# Autodesk Inventor assembly: Assembly - Main
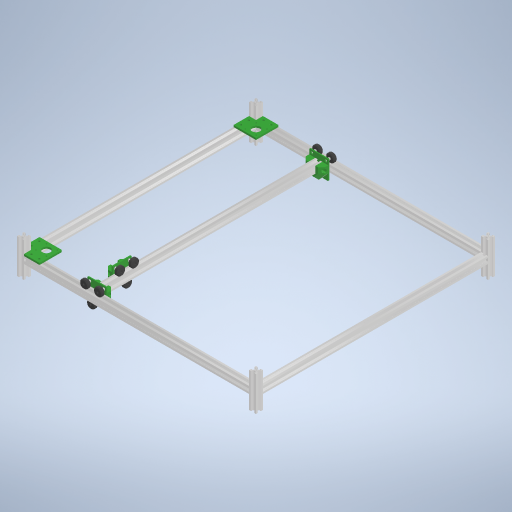
[picture p0: Inventor's stored thumbnail of the model, 512x512]
Saved by Autodesk Inventor 2023 (Build 270158000, 158)
## iProperties
Created: 2023-04-10
Part Number: Assembly - Main
Document SubType Name: Assembly
Designer: ethan
Author: ethan
## Documents named in this file (6)
- C:\Users\ethan\Documents\GitHub\WU-AutomaticChessboard\CAD\Assembly - Main.iam
- C:\Users\ethan\Documents\GitHub\WU-AutomaticChessboard\CAD\VSlot Extrusion 20x20x650mm.ipt
- C:\Users\ethan\Documents\GitHub\WU-AutomaticChessboard\CAD\VSlot Extrusion 20x20x100mm.ipt
- C:\Users\ethan\Documents\GitHub\WU-AutomaticChessboard\CAD\Assembly - GantryPlate.iam
- C:\Users\ethan\Documents\GitHub\WU-AutomaticChessboard\CAD\VSlot Extrusion 20x20x637,50mm.ipt
- C:\Users\ethan\Documents\GitHub\WU-AutomaticChessboard\CAD\NEMA17 Stepper CornerMount.ipt
## Components (14 placed, 5 different names)
1. VSlot Extrusion 20x20x650mm:1 — Flush:1, Mate:1, Flush:2, Flush:5, Mate:3, Flush:6, Flush:15, Tangent:3, Tangent:4, Tangent:6, Flush:22
2. VSlot Extrusion 20x20x650mm:2 — Mate:2, Flush:3, Flush:4, Mate:4, Flush:7, Flush:14
3. VSlot Extrusion 20x20x650mm:3 — Mate:8, Flush:12, Flush:13, Flush:20, Mate:13, Flush:21, Mate:14
4. VSlot Extrusion 20x20x650mm:4 — Mate:6, Flush:8, Flush:9, Mate:7, Flush:10, Flush:11, Mate:9, Tangent:1, Tangent:2, Tangent:5, Flush:19
5. VSlot Extrusion 20x20x100mm:1 — Mate:7, Flush:10, Flush:11, Mate:8, Flush:12, Flush:13
6. VSlot Extrusion 20x20x100mm:2 — Mate:4, Flush:7, Mate:6, Flush:8, Flush:9, Flush:14
7. VSlot Extrusion 20x20x100mm:3 — Flush:5, Mate:3, Flush:6
8. VSlot Extrusion 20x20x100mm:4 — Flush:1, Mate:1, Flush:2, Mate:2, Flush:3, Flush:4
9. Assembly - GantryPlate:1 [sub-assembly] — Mate:9, Tangent:1, Tangent:2, Tangent:5, Mate:12, Flush:17
10. Assembly - GantryPlate:2 [sub-assembly] — Flush:15, Tangent:3, Tangent:4, Tangent:6, Mate:10, Mate:11, Flush:16
11. VSlot Extrusion 20x20x637,50mm:1 — Mate:10, Mate:11, Flush:16, Mate:12, Flush:17, Flush:18, Tangent:7, Tangent:8, Tangent:9
12. Assembly - GantryPlate:3 [sub-assembly] — Flush:18, Tangent:7, Tangent:8, Tangent:9
13. NEMA17 Stepper CornerMount:1 — Flush:19, Flush:20, Mate:13
14. NEMA17 Stepper CornerMount:2 — Flush:21, Flush:22, Mate:14
## Relationships (44: Flush 22, Mate 13, Tangent 9)
- Flush:1: VSlot Extrusion 20x20x650mm:1 ↔ VSlot Extrusion 20x20x100mm:4
- Mate:1: VSlot Extrusion 20x20x650mm:1 ↔ VSlot Extrusion 20x20x100mm:4
- Flush:2 (-40 mm): VSlot Extrusion 20x20x650mm:1 ↔ VSlot Extrusion 20x20x100mm:4
- Mate:2: VSlot Extrusion 20x20x650mm:2 ↔ VSlot Extrusion 20x20x100mm:4
- Flush:3: VSlot Extrusion 20x20x650mm:2 ↔ VSlot Extrusion 20x20x100mm:4
- Flush:4 (-40 mm): VSlot Extrusion 20x20x650mm:2 ↔ VSlot Extrusion 20x20x100mm:4
- Flush:5: VSlot Extrusion 20x20x650mm:1 ↔ VSlot Extrusion 20x20x100mm:3
- Mate:3: VSlot Extrusion 20x20x650mm:1 ↔ VSlot Extrusion 20x20x100mm:3
- Flush:6 (-40 mm): VSlot Extrusion 20x20x650mm:1 ↔ VSlot Extrusion 20x20x100mm:3
- Mate:4: VSlot Extrusion 20x20x650mm:2 ↔ VSlot Extrusion 20x20x100mm:2
- Flush:7: VSlot Extrusion 20x20x650mm:2 ↔ VSlot Extrusion 20x20x100mm:2
- Mate:6: VSlot Extrusion 20x20x650mm:4 ↔ VSlot Extrusion 20x20x100mm:2
- Flush:8: VSlot Extrusion 20x20x650mm:4 ↔ VSlot Extrusion 20x20x100mm:2
- Flush:9 (-40 mm): VSlot Extrusion 20x20x650mm:4 ↔ VSlot Extrusion 20x20x100mm:2
- Mate:7: VSlot Extrusion 20x20x650mm:4 ↔ VSlot Extrusion 20x20x100mm:1
- Flush:10: VSlot Extrusion 20x20x650mm:4 ↔ VSlot Extrusion 20x20x100mm:1
- Flush:11 (-40 mm): VSlot Extrusion 20x20x650mm:4 ↔ VSlot Extrusion 20x20x100mm:1
- Mate:8: VSlot Extrusion 20x20x650mm:3 ↔ VSlot Extrusion 20x20x100mm:1
- Flush:12: VSlot Extrusion 20x20x650mm:3 ↔ VSlot Extrusion 20x20x100mm:1
- Flush:13 (-40 mm): VSlot Extrusion 20x20x650mm:3 ↔ VSlot Extrusion 20x20x100mm:1
- Flush:14 (-40 mm): VSlot Extrusion 20x20x650mm:2 ↔ VSlot Extrusion 20x20x100mm:2
- Mate:9 (-5.25 mm): VSlot Extrusion 20x20x650mm:4 ↔ Assembly - GantryPlate:1
- Tangent:1: VSlot Extrusion 20x20x650mm:4 ↔ Assembly - GantryPlate:1
- Tangent:2: VSlot Extrusion 20x20x650mm:4 ↔ Assembly - GantryPlate:1
- Flush:15 (23.25 mm): VSlot Extrusion 20x20x650mm:1 ↔ Assembly - GantryPlate:2
- Tangent:3: VSlot Extrusion 20x20x650mm:1 ↔ Assembly - GantryPlate:2
- Tangent:4: VSlot Extrusion 20x20x650mm:1 ↔ Assembly - GantryPlate:2
- Tangent:5: VSlot Extrusion 20x20x650mm:4 ↔ Assembly - GantryPlate:1
- Tangent:6: VSlot Extrusion 20x20x650mm:1 ↔ Assembly - GantryPlate:2
- Mate:10: Assembly - GantryPlate:2 ↔ VSlot Extrusion 20x20x637,50mm:1
- Mate:11: Assembly - GantryPlate:2 ↔ VSlot Extrusion 20x20x637,50mm:1
- Flush:16: Assembly - GantryPlate:2 ↔ VSlot Extrusion 20x20x637,50mm:1
- Mate:12: Assembly - GantryPlate:1 ↔ VSlot Extrusion 20x20x637,50mm:1
- Flush:17: Assembly - GantryPlate:1 ↔ VSlot Extrusion 20x20x637,50mm:1
- Flush:18 (23.25 mm): VSlot Extrusion 20x20x637,50mm:1 ↔ Assembly - GantryPlate:3
- Tangent:7: VSlot Extrusion 20x20x637,50mm:1 ↔ Assembly - GantryPlate:3
- Tangent:8: VSlot Extrusion 20x20x637,50mm:1 ↔ Assembly - GantryPlate:3
- Tangent:9: VSlot Extrusion 20x20x637,50mm:1 ↔ Assembly - GantryPlate:3
- Flush:19: VSlot Extrusion 20x20x650mm:4 ↔ NEMA17 Stepper CornerMount:1
- Flush:20: VSlot Extrusion 20x20x650mm:3 ↔ NEMA17 Stepper CornerMount:1
- Mate:13: VSlot Extrusion 20x20x650mm:3 ↔ NEMA17 Stepper CornerMount:1
- Flush:21: VSlot Extrusion 20x20x650mm:3 ↔ NEMA17 Stepper CornerMount:2
- Flush:22: VSlot Extrusion 20x20x650mm:1 ↔ NEMA17 Stepper CornerMount:2
- Mate:14: VSlot Extrusion 20x20x650mm:3 ↔ NEMA17 Stepper CornerMount:2
